# Autodesk Inventor assembly: BHSS
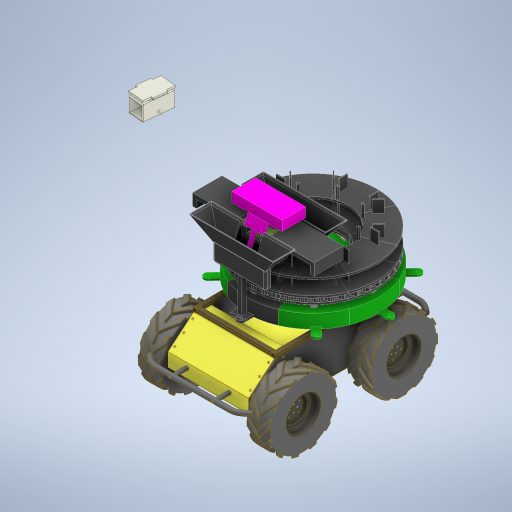
[picture p0: Inventor's stored thumbnail of the model, 512x512]
Saved by Autodesk Inventor 2023 (Build 270158000, 158)
## iProperties
Created: 2022-10-26
Part Number: BHSS
Document SubType Name: Assembly
Designer: cheng
Mass: 107138 g
Surface Area: 105016 cm^2
Volume: 89092.4 cm^3
Density: 1.20255 g/cm^3
Author: cheng
## Documents named in this file (11)
- C:\Users\mihal\Desktop\4th Year Project\BHSS DESIGN\Sixth Assembly\BHSS.iam
- C:\Users\mihal\Desktop\4th Year Project\BHSS DESIGN\Sixth Assembly\Battery Cage.ipt
- C:\Users\mihal\Desktop\4th Year Project\BHSS DESIGN\Sixth Assembly\Battery Container.ipt
- C:\Users\mihal\Desktop\4th Year Project\BHSS DESIGN\Sixth Assembly\Box Base Plate.ipt
- C:\Users\mihal\Desktop\4th Year Project\BHSS DESIGN\Sixth Assembly\Carousel Fixed Track.ipt
- C:\Users\mihal\Desktop\4th Year Project\BHSS DESIGN\Sixth Assembly\drone model.ipt
- C:\Users\mihal\Desktop\4th Year Project\BHSS DESIGN\Sixth Assembly\Husky_3D_Model.ipt
- C:\Users\mihal\Desktop\4th Year Project\BHSS DESIGN\Sixth Assembly\Landing dock V2.ipt
- C:\Users\mihal\Desktop\4th Year Project\BHSS DESIGN\Sixth Assembly\Battery Cage Spring Plate.ipt
- C:\Users\mihal\Desktop\4th Year Project\BHSS DESIGN\Sixth Assembly\Inner Circle Landing Legs.ipt
- C:\Users\mihal\Desktop\4th Year Project\BHSS DESIGN\Sixth Assembly\Full Roller Carousel Assembly.iam
## Components (18 placed, 10 different names)
1. Box Base Plate:1 — Mate:4, Mate:5, Mate:6, Mate:18, Mate:19, Mate:20, Mate:25, Flush:1, Mate:107, Mate:110, Mate:111, Mate:117, Mate:118
2. Carousel Fixed Track:1 — Mate:4, Mate:10, Mate:11
3. Carousel Fixed Track:2 — Mate:5, Mate:14, Mate:15, Mate:16, Mate:17, Mate:119
4. Carousel Fixed Track:3 — Mate:10, Mate:11, Mate:12, Mate:13, Mate:25, Angle:1
5. Carousel Fixed Track:4 — Mate:6, Mate:12, Mate:13, Mate:14, Mate:15, Mate:120
6. Carousel Fixed Track:5 — Mate:16, Mate:17, Mate:18, Mate:21, Mate:22
7. Carousel Fixed Track:6 — Mate:19, Mate:23, Mate:24, Mate:108, Mate:109
8. Carousel Fixed Track:7 — Mate:20, Mate:21, Mate:22, Mate:23, Mate:24
9. drone model:1 — Mate:114, Mate:115, Mate:116
10. Husky_3D_Model:1 — Flush:1
11. Battery Container:19
12. Carousel Fixed Track:8 — Mate:107, Mate:108, Mate:109
13. Landing dock V2:1 — Mate:110, Mate:111
14. Battery Cage:1 — Mate:112, Mate:113, Mate:114, Mate:115, Mate:116
15. Battery Cage Spring Plate:2 — Mate:112, Mate:113
16. Inner Circle Landing Legs:2 — Mate:117
17. Inner Circle Landing Legs:4 — Mate:118
18. Full Roller Carousel Assembly:1 [sub-assembly] — Mate:119, Mate:120, Angle:1
## Relationships (35: Mate 33, Flush 1, Angle 1)
- Mate:4: Box Base Plate:1 ↔ Carousel Fixed Track:1
- Mate:5: Box Base Plate:1 ↔ Carousel Fixed Track:2
- Mate:6: Box Base Plate:1 ↔ Carousel Fixed Track:4
- Mate:10: Carousel Fixed Track:1 ↔ Carousel Fixed Track:3
- Mate:11: Carousel Fixed Track:1 ↔ Carousel Fixed Track:3
- Mate:12: Carousel Fixed Track:3 ↔ Carousel Fixed Track:4
- Mate:13: Carousel Fixed Track:3 ↔ Carousel Fixed Track:4
- Mate:14: Carousel Fixed Track:2 ↔ Carousel Fixed Track:4
- Mate:15: Carousel Fixed Track:2 ↔ Carousel Fixed Track:4
- Mate:16: Carousel Fixed Track:2 ↔ Carousel Fixed Track:5
- Mate:17: Carousel Fixed Track:2 ↔ Carousel Fixed Track:5
- Mate:18: Box Base Plate:1 ↔ Carousel Fixed Track:5
- Mate:19: Box Base Plate:1 ↔ Carousel Fixed Track:6
- Mate:20: Box Base Plate:1 ↔ Carousel Fixed Track:7
- Mate:21: Carousel Fixed Track:5 ↔ Carousel Fixed Track:7
- Mate:22: Carousel Fixed Track:5 ↔ Carousel Fixed Track:7
- Mate:23: Carousel Fixed Track:6 ↔ Carousel Fixed Track:7
- Mate:24: Carousel Fixed Track:6 ↔ Carousel Fixed Track:7
- Mate:25: Box Base Plate:1 ↔ Carousel Fixed Track:3
- Flush:1: Box Base Plate:1 ↔ Husky_3D_Model:1
- Mate:107: Box Base Plate:1 ↔ Carousel Fixed Track:8
- Mate:108: Carousel Fixed Track:6 ↔ Carousel Fixed Track:8
- Mate:109: Carousel Fixed Track:6 ↔ Carousel Fixed Track:8
- Mate:110: Box Base Plate:1 ↔ Landing dock V2:1
- Mate:111: Box Base Plate:1 ↔ Landing dock V2:1
- Mate:112: Battery Cage:1 ↔ Battery Cage Spring Plate:2
- Mate:113: Battery Cage:1 ↔ Battery Cage Spring Plate:2
- Mate:114: drone model:1 ↔ Battery Cage:1
- Mate:115: drone model:1 ↔ Battery Cage:1
- Mate:116: drone model:1 ↔ Battery Cage:1
- Mate:117: Box Base Plate:1 ↔ Inner Circle Landing Legs:2
- Mate:118: Box Base Plate:1 ↔ Inner Circle Landing Legs:4
- Mate:119: Carousel Fixed Track:2 ↔ Full Roller Carousel Assembly:1
- Mate:120: Carousel Fixed Track:4 ↔ Full Roller Carousel Assembly:1
- Angle:1 (0 deg): Carousel Fixed Track:3 ↔ Full Roller Carousel Assembly:1
